# Autodesk Inventor assembly: sub_leg_1
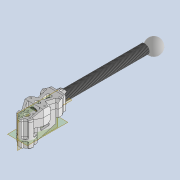
[picture p0: Inventor's stored thumbnail of the model, 180x180]
Saved by Autodesk Inventor 2020 (Build 240168000, 168)
## iProperties
Created: 2020-08-29
Part Number: sub_leg_1
Document SubType Name: Assembly
Designer: psrobotics
Author: psrobotics
## Documents named in this file (6)
- E:\projects-3\biped_gen1\hardware\sub_leg_1.iam
- E:\projects-3\biped_gen1\hardware\carbon_fiber_25_21_300.ipt
- E:\projects-3\biped_gen1\hardware\joint_connector_4.ipt
- E:\projects-3\biped_gen1\hardware\joint_connector_5.ipt
- E:\projects-3\biped_gen1\hardware\joint_connector_6.ipt
- E:\projects-3\biped_gen1\hardware\legend_40mm.ipt
## Components (5 placed, 5 different names)
1. carbon_fiber_25_21_300:1 — Flush:1, Insert:1, Tangent:1
2. joint_connector_4:1 — Flush:1, Insert:1, Insert:2, Insert:3, Insert:4
3. joint_connector_6:1 — Insert:4, Insert:5
4. joint_connector_5:1 — Insert:2, Insert:3, Insert:5
5. legend_40mm:1 — Tangent:1
## Relationships (7: Insert 5, Flush 1, Tangent 1)
- Flush:1: carbon_fiber_25_21_300:1 ↔ joint_connector_4:1
- Insert:1: carbon_fiber_25_21_300:1 ↔ joint_connector_4:1
- Insert:2: joint_connector_4:1 ↔ joint_connector_5:1
- Insert:3: joint_connector_4:1 ↔ joint_connector_5:1
- Insert:4: joint_connector_4:1 ↔ joint_connector_6:1
- Insert:5: joint_connector_6:1 ↔ joint_connector_5:1
- Tangent:1: carbon_fiber_25_21_300:1 ↔ legend_40mm:1
